# Autodesk Inventor assembly: s-assy-odrive
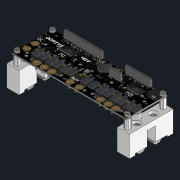
[picture p0: Inventor's stored thumbnail of the model, 180x180]
Saved by Autodesk Inventor 2022 (Build 260153000, 153)
## iProperties
Created: 2021-10-21
Part Number: s-assy-odrive
Document SubType Name: Assembly
Designer: Yuta Kage
Author: Yuta Kage
## Documents named in this file (8)
- C:\Users\yuta0\Documents\GitHub\catchrobo_hardware\assy-scara\s-assy-odrive.iam
- C:\Users\yuta0\Documents\GitHub\catchrobo_hardware\assy-scara\ODrive3.4.ipt
- C:\Users\yuta0\Documents\GitHub\catchrobo_hardware\assy-scara\scara-base7.ipt
- C:\Users\yuta0\Documents\GitHub\catchrobo_hardware\assy-scara\SB-305060.ipt
- C:\Users\yuta0\Documents\GitHub\catchrobo_hardware\assy-scara\hexagonal_spacer_M3_12mm.ipt
- C:\Users\yuta0\Documents\GitHub\catchrobo_hardware\assy-scara\CB5-22.ipt
- C:\Users\yuta0\Documents\GitHub\catchrobo_hardware\assy-scara\HNTT5-5.ipt
- C:\Users\yuta0\Documents\GitHub\catchrobo_hardware\assy-scara\CB3-5.ipt
## Components (23 placed, 7 different names)
1. ODrive3.4:1 — メイト:1, メイト:2, メイト:6, メイト:12, メイト:13
2. scara-base7:1 — メイト:1, メイト:2, メイト:3, フラッシュ:1, メイト:5, メイト:7, メイト:8, メイト:9, メイト:11, 角度:1
3. scara-base7:2
4. hexagonal_spacer_M3_12mm:1 — メイト:4, メイト:5, メイト:6
5. SB-305060:1 — メイト:3, フラッシュ:1, メイト:4
6. CB3-5:1 — メイト:12, メイト:13
7. hexagonal_spacer_M3_12mm:2
8. SB-305060:2
9. CB3-5:2
10. CB5-22:1 — メイト:7, メイト:8, メイト:9, メイト:10
11. HNTT5-5:1 — メイト:10, メイト:11, 角度:1
12. CB5-22:2
13. HNTT5-5:2
14. hexagonal_spacer_M3_12mm:3
15. SB-305060:3
16. CB3-5:3
17. hexagonal_spacer_M3_12mm:4
18. SB-305060:4
19. CB3-5:4
20. CB5-22:3
21. HNTT5-5:3
22. CB5-22:4
23. HNTT5-5:4
## Component patterns: (2 elements, first: scara-base7:1), (2 elements, first: hexagonal_spacer_M3_12mm:1 + SB-305060:1 + CB3-5:1), (2 elements, first: CB5-22:1 + HNTT5-5:1), コンポーネント パターン 1:2 (2 elements), コンポーネント パターン 2:2 (2 elements)
## Relationships (15: Mate 13, Flush 1, Angle 1)
- メイト:1 [Mate]: ODrive3.4:1 ↔ scara-base7:1
- メイト:2 [Mate]: ODrive3.4:1 ↔ scara-base7:1
- メイト:3 [Mate]: scara-base7:1 ↔ SB-305060:1
- フラッシュ:1 [Flush]: scara-base7:1 ↔ SB-305060:1
- メイト:4 [Mate]: hexagonal_spacer_M3_12mm:1 ↔ SB-305060:1
- メイト:5 [Mate]: scara-base7:1 ↔ hexagonal_spacer_M3_12mm:1
- メイト:6 [Mate]: ODrive3.4:1 ↔ hexagonal_spacer_M3_12mm:1
- メイト:7 [Mate]: scara-base7:1 ↔ CB5-22:1
- メイト:8 [Mate]: scara-base7:1 ↔ CB5-22:1
- メイト:9 [Mate]: scara-base7:1 ↔ CB5-22:1
- メイト:10 [Mate]: CB5-22:1 ↔ HNTT5-5:1
- メイト:11 [Mate] (2 mm): scara-base7:1 ↔ HNTT5-5:1
- 角度:1 [Angle] (0 deg): scara-base7:1 ↔ HNTT5-5:1
- メイト:12 [Mate]: ODrive3.4:1 ↔ CB3-5:1
- メイト:13 [Mate]: ODrive3.4:1 ↔ CB3-5:1
